# Autodesk Inventor assembly: Base-soporte
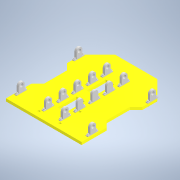
[picture p0: Inventor's stored thumbnail of the model, 180x180]
Saved by Autodesk Inventor 2021 (Build 250183000, 183)
## iProperties
Created: 2021-02-07
Part Number: Base-soporte
Document SubType Name: Assembly
Designer: rotje
Author: rotje
## Documents named in this file (5)
- C:\Users\rotje\Documents\Inventor\MSF\Base-soporte.iam
- C:\Users\rotje\Documents\Inventor\MSF\BaseCarro.ipt
- C:\Users\rotje\Documents\Inventor\MSF\sopoetellantas.ipt
- C:\Users\rotje\Documents\Inventor\MSF\soporte_para_engrane.ipt
- C:\Users\rotje\Documents\Inventor\MSF\din_912-m5x0_8-20-8_8.ipt
## Components (43 placed, 4 different names)
1. BaseCarro:1 — Insertar:1, Insertar:2, Insertar:3, Insertar:4, Insertar:5, Insertar:6, Insertar:7, Insertar:8, Insertar:11, Insertar:12, Insertar:13, Insertar:14, Insertar:15, Insertar:16, Insertar:21, Insertar:22, Insertar:23, Insertar:24, Insertar:25, Insertar:26, Insertar:57, Insertar:58, Insertar:59, Insertar:60, Insertar:61, Insertar:62, Insertar:63, Insertar:64
2. sopoetellantas:1 — Insertar:1, Insertar:2, Insertar:29, Insertar:30
3. sopoetellantas:2 — Insertar:7, Insertar:8, Insertar:53, Insertar:54
4. sopoetellantas:3 — Insertar:3, Insertar:4, Insertar:31, Insertar:32
5. sopoetellantas:4 — Insertar:5, Insertar:6, Insertar:55, Insertar:56
6. soporte_para_engrane:2 — Insertar:15, Insertar:16, Insertar:35, Insertar:36
7. soporte_para_engrane:3 — Insertar:13, Insertar:14, Insertar:37, Insertar:38
8. soporte_para_engrane:4 — Insertar:11, Insertar:12, Insertar:39, Insertar:40
9. soporte_para_engrane:7 — Insertar:25, Insertar:26, Insertar:49, Insertar:50
10. soporte_para_engrane:8 — Insertar:23, Insertar:24, Insertar:45, Insertar:46
11. soporte_para_engrane:9 — Insertar:21, Insertar:22, Insertar:47, Insertar:48
12. din_912-m5x0_8-20-8_8:1 — Insertar:29
13. din_912-m5x0_8-20-8_8:2 — Insertar:69
14. din_912-m5x0_8-20-8_8:3 — Insertar:32
15. din_912-m5x0_8-20-8_8:4 — Insertar:31
16. din_912-m5x0_8-20-8_8:5 — Insertar:53
17. din_912-m5x0_8-20-8_8:6 — Insertar:54
18. din_912-m5x0_8-20-8_8:7 — Insertar:66
19. din_912-m5x0_8-20-8_8:8 — Insertar:65
20. din_912-m5x0_8-20-8_8:9 — Insertar:46
21. din_912-m5x0_8-20-8_8:10 — Insertar:45
22. din_912-m5x0_8-20-8_8:11 — Insertar:50
23. din_912-m5x0_8-20-8_8:12 — Insertar:49
24. din_912-m5x0_8-20-8_8:15 — Insertar:56
25. din_912-m5x0_8-20-8_8:16 — Insertar:71
26. din_912-m5x0_8-20-8_8:17 — Insertar:47
27. din_912-m5x0_8-20-8_8:18 — Insertar:48
28. din_912-m5x0_8-20-8_8:19 — Insertar:72
29. din_912-m5x0_8-20-8_8:20 — Insertar:55
30. din_912-m5x0_8-20-8_8:21 — Insertar:30
31. din_912-m5x0_8-20-8_8:22 — Insertar:70
32. din_912-m5x0_8-20-8_8:23 — Insertar:35
33. din_912-m5x0_8-20-8_8:24 — Insertar:36
34. din_912-m5x0_8-20-8_8:25 — Insertar:37
35. din_912-m5x0_8-20-8_8:26 — Insertar:38
36. din_912-m5x0_8-20-8_8:27 — Insertar:39
37. din_912-m5x0_8-20-8_8:28 — Insertar:40
38. din_912-m5x0_8-20-8_8:29 — Insertar:67
39. din_912-m5x0_8-20-8_8:30 — Insertar:68
40. sopoetellantas:5 — Insertar:57, Insertar:58, Insertar:69, Insertar:70
41. sopoetellantas:6 — Insertar:59, Insertar:60, Insertar:71, Insertar:72
42. sopoetellantas:7 — Insertar:63, Insertar:64, Insertar:65, Insertar:66
43. sopoetellantas:8 — Insertar:61, Insertar:62, Insertar:67, Insertar:68
## Relationships (56: Insert 56)
- Insertar:1: BaseCarro:1 ↔ sopoetellantas:1
- Insertar:2: BaseCarro:1 ↔ sopoetellantas:1
- Insertar:3: BaseCarro:1 ↔ sopoetellantas:3
- Insertar:4: BaseCarro:1 ↔ sopoetellantas:3
- Insertar:5: BaseCarro:1 ↔ sopoetellantas:4
- Insertar:6: BaseCarro:1 ↔ sopoetellantas:4
- Insertar:7: BaseCarro:1 ↔ sopoetellantas:2
- Insertar:8: BaseCarro:1 ↔ sopoetellantas:2
- Insertar:11: BaseCarro:1 ↔ soporte_para_engrane:4
- Insertar:12: BaseCarro:1 ↔ soporte_para_engrane:4
- Insertar:13: BaseCarro:1 ↔ soporte_para_engrane:3
- Insertar:14: BaseCarro:1 ↔ soporte_para_engrane:3
- Insertar:15: BaseCarro:1 ↔ soporte_para_engrane:2
- Insertar:16: BaseCarro:1 ↔ soporte_para_engrane:2
- Insertar:21: BaseCarro:1 ↔ soporte_para_engrane:9
- Insertar:22: BaseCarro:1 ↔ soporte_para_engrane:9
- Insertar:23: BaseCarro:1 ↔ soporte_para_engrane:8
- Insertar:24: BaseCarro:1 ↔ soporte_para_engrane:8
- Insertar:25: BaseCarro:1 ↔ soporte_para_engrane:7
- Insertar:26: BaseCarro:1 ↔ soporte_para_engrane:7
- Insertar:29: sopoetellantas:1 ↔ din_912-m5x0_8-20-8_8:1
- Insertar:30: sopoetellantas:1 ↔ din_912-m5x0_8-20-8_8:21
- Insertar:31: sopoetellantas:3 ↔ din_912-m5x0_8-20-8_8:4
- Insertar:32: sopoetellantas:3 ↔ din_912-m5x0_8-20-8_8:3
- Insertar:35: soporte_para_engrane:2 ↔ din_912-m5x0_8-20-8_8:23
- Insertar:36: soporte_para_engrane:2 ↔ din_912-m5x0_8-20-8_8:24
- Insertar:37: soporte_para_engrane:3 ↔ din_912-m5x0_8-20-8_8:25
- Insertar:38: soporte_para_engrane:3 ↔ din_912-m5x0_8-20-8_8:26
- Insertar:39: soporte_para_engrane:4 ↔ din_912-m5x0_8-20-8_8:27
- Insertar:40: soporte_para_engrane:4 ↔ din_912-m5x0_8-20-8_8:28
- Insertar:45: soporte_para_engrane:8 ↔ din_912-m5x0_8-20-8_8:10
- Insertar:46: soporte_para_engrane:8 ↔ din_912-m5x0_8-20-8_8:9
- Insertar:47: soporte_para_engrane:9 ↔ din_912-m5x0_8-20-8_8:17
- Insertar:48: soporte_para_engrane:9 ↔ din_912-m5x0_8-20-8_8:18
- Insertar:49: soporte_para_engrane:7 ↔ din_912-m5x0_8-20-8_8:12
- Insertar:50: soporte_para_engrane:7 ↔ din_912-m5x0_8-20-8_8:11
- Insertar:53: sopoetellantas:2 ↔ din_912-m5x0_8-20-8_8:5
- Insertar:54: sopoetellantas:2 ↔ din_912-m5x0_8-20-8_8:6
- Insertar:55: sopoetellantas:4 ↔ din_912-m5x0_8-20-8_8:20
- Insertar:56: sopoetellantas:4 ↔ din_912-m5x0_8-20-8_8:15
- Insertar:57: BaseCarro:1 ↔ sopoetellantas:5
- Insertar:58: BaseCarro:1 ↔ sopoetellantas:5
- Insertar:59: BaseCarro:1 ↔ sopoetellantas:6
- Insertar:60: BaseCarro:1 ↔ sopoetellantas:6
- Insertar:61: BaseCarro:1 ↔ sopoetellantas:8
- Insertar:62: BaseCarro:1 ↔ sopoetellantas:8
- Insertar:63: BaseCarro:1 ↔ sopoetellantas:7
- Insertar:64: BaseCarro:1 ↔ sopoetellantas:7
- Insertar:65: din_912-m5x0_8-20-8_8:8 ↔ sopoetellantas:7
- Insertar:66: din_912-m5x0_8-20-8_8:7 ↔ sopoetellantas:7
- Insertar:67: din_912-m5x0_8-20-8_8:29 ↔ sopoetellantas:8
- Insertar:68: din_912-m5x0_8-20-8_8:30 ↔ sopoetellantas:8
- Insertar:69: din_912-m5x0_8-20-8_8:2 ↔ sopoetellantas:5
- Insertar:70: din_912-m5x0_8-20-8_8:22 ↔ sopoetellantas:5
- Insertar:71: din_912-m5x0_8-20-8_8:16 ↔ sopoetellantas:6
- Insertar:72: din_912-m5x0_8-20-8_8:19 ↔ sopoetellantas:6
